# Autodesk Inventor assembly: Assembly1
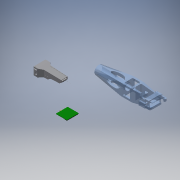
[picture p0: Inventor's stored thumbnail of the model, 180x180]
Saved by Autodesk Inventor 2019 (Build 230136000, 136)
## iProperties
Created: 2020-03-26
Part Number: Assembly1
Document SubType Name: Assembly
Designer: Thomas Zhihao Luo
Mass: 8.78558 g
Surface Area: 110.094 cm^2
Volume: 8.78558 cm^3
Density: 1 g/cm^3
Author: Thomas Zhihao Luo
## Documents named in this file (8)
- C:\Users\Thomas Zhihao Luo\Documents\chronic_neuropixels\2.611\Assembly1.iam
- C:\Users\Thomas Zhihao Luo\Documents\chronic_neuropixels\2.611\external_bottom.ipt
- C:\Users\Thomas Zhihao Luo\Documents\chronic_neuropixels\2.611\external_top.ipt
- C:\Users\Thomas Zhihao Luo\Documents\chronic_neuropixels\2.611\headstage.ipt
- C:\Users\Thomas Zhihao Luo\Documents\chronic_neuropixels\2.611\headstage_mount.ipt
- C:\Users\Thomas Zhihao Luo\Documents\chronic_neuropixels\2.611\probe.ipt
- C:\Users\Thomas Zhihao Luo\Documents\chronic_neuropixels\2.611\base.ipt
- C:\Users\Thomas Zhihao Luo\Documents\chronic_neuropixels\2.611\holder.ipt
## Components (7 placed, 7 different names)
1. external_bottom:1 — Rotational:1, Mate:4, Mate:5
2. external_top:1 — Mate:4, Mate:5
3. headstage:1
4. headstage_mount:1
5. probe:1 — Mate:1, Flush:1, Mate:2
6. base:1 — Mate:1, Flush:1, Mate:2, Mate:3, Flush:2, Flush:3
7. holder:1 — Mate:3, Flush:2, Flush:3, Rotational:1
## Relationships (9: Mate 5, Flush 3, RevoluteJoint 1)
- Mate:1: probe:1 ↔ base:1
- Flush:1: probe:1 ↔ base:1
- Mate:2: probe:1 ↔ base:1
- Mate:3: base:1 ↔ holder:1
- Flush:2: base:1 ↔ holder:1
- Flush:3: base:1 ↔ holder:1
- Rotational:1 [RevoluteJoint]: external_bottom:1 ↔ holder:1
- Mate:4: external_bottom:1 ↔ external_top:1
- Mate:5: external_bottom:1 ↔ external_top:1
